# Autodesk Inventor assembly: Ensamblaje2
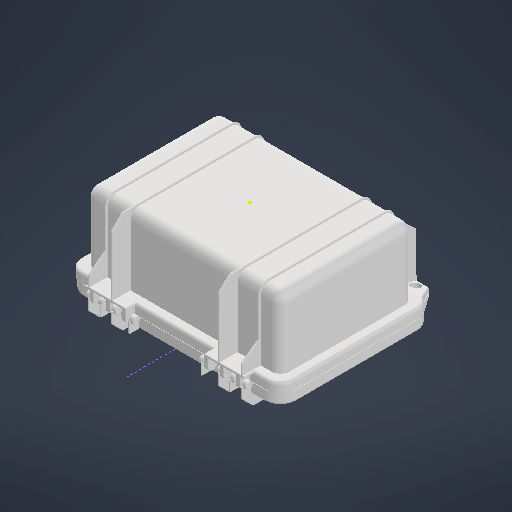
[picture p0: Inventor's stored thumbnail of the model, 512x512]
Saved by Autodesk Inventor 2026.2 (Build 302298000, 298)
## iProperties
Created: 2026-01-07
Part Number: Ensamblaje2
Document SubType Name: Assembly
Designer: vicho
Author: vicho
## Documents named in this file (3)
- C:\Users\vicho\OneDrive\Documentos\MODELACION PROYECTOS\Caja de componentes\Ensamblaje2.iam
- C:\Users\vicho\OneDrive\Documentos\PROYECTOS INVENTOR\caja componentes\caja.ipt
- C:\Users\vicho\OneDrive\Documentos\PROYECTOS INVENTOR\caja componentes\tapa caja.ipt
## Components (2 placed, 2 different names)
1. caja:2 — Nivelación:1, Nivelación:2, Nivelación:3, Coincidencia:1, Coincidencia:2
2. tapa caja:1 — Coincidencia:1, Coincidencia:2
## Relationships (5: Flush 3, Mate 2)
- Nivelación:1 [Flush]: caja:2
- Nivelación:2 [Flush]: caja:2
- Nivelación:3 [Flush]: caja:2
- Coincidencia:1 [Mate]: caja:2 ↔ tapa caja:1
- Coincidencia:2 [Mate] (0.05 mm): caja:2 ↔ tapa caja:1
